# Autodesk Inventor assembly: Assembly19
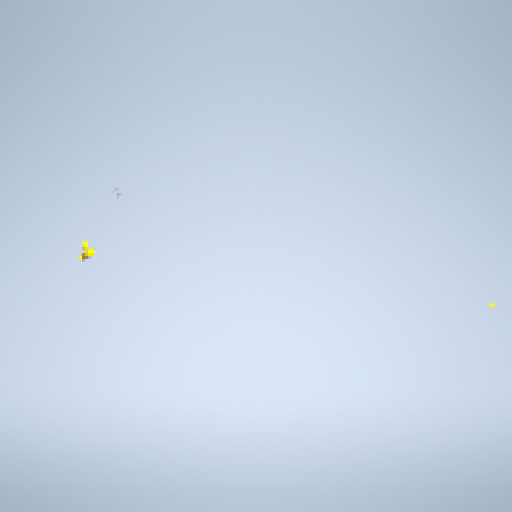
[picture p0: Inventor's stored thumbnail of the model, 512x512]
Saved by Autodesk Inventor 2024.1 (Build 281209000, 209)
## iProperties
Created: 2023-11-10
Part Number: Assembly19
Document SubType Name: Assembly
Designer: luvag
Author: luvag
## Documents named in this file (4)
- C:\Users\luvag\Desktop\Assembly19.iam
- C:\Users\luvag\Desktop\Assembly15.iam
- C:\Users\luvag\Desktop\eg part 1.ipt
- C:\Users\luvag\Desktop\rod.ipt
## Components (3 placed, 3 different names)
1. Assembly15:1 [sub-assembly]
2. eg part 1:1
3. rod:1
## Relationships (1: Transitional 1)
- [Transitional]: Assembly15:1 ↔ rod:1
